# Autodesk Inventor assembly: Koło_przednie
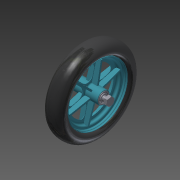
[picture p0: Inventor's stored thumbnail of the model, 180x180]
Saved by Autodesk Inventor 2015 (Build 190159000, 159)
## iProperties
Created: 2015-12-01
Part Number: Koło_przednie
Document SubType Name: Assembly
Designer: graaapsik
Author: graaapsik
## Documents named in this file (7)
- C:\Users\EriveltonDell\Documents\Centro Universitário da FEI\Wheelchair\CADEIRA DE RODAS - DESENHO\lasteverision\Power-Assisted-Wheelchair-master\Koło_przednie.iam
- C:\Users\EriveltonDell\Documents\Centro Universitário da FEI\Wheelchair\CADEIRA DE RODAS - DESENHO\lasteverision\Power-Assisted-Wheelchair-master\Obręcz_koła_przedniego.ipt
- C:\Users\EriveltonDell\Documents\Centro Universitário da FEI\Wheelchair\CADEIRA DE RODAS - DESENHO\lasteverision\Power-Assisted-Wheelchair-master\ISO 4016 - M8 x 65.ipt
- C:\Users\EriveltonDell\Documents\Centro Universitário da FEI\Wheelchair\CADEIRA DE RODAS - DESENHO\lasteverision\Power-Assisted-Wheelchair-master\ISO 4032 - M8ISO.ipt
- C:\Users\EriveltonDell\Documents\Centro Universitário da FEI\Wheelchair\CADEIRA DE RODAS - DESENHO\lasteverision\Power-Assisted-Wheelchair-master\Rolling bearing 70000B S719_8 GB_T 292-94.ipt
- C:\Users\EriveltonDell\Documents\Centro Universitário da FEI\Wheelchair\CADEIRA DE RODAS - DESENHO\lasteverision\Power-Assisted-Wheelchair-master\Separator.ipt
- C:\Users\EriveltonDell\Documents\Centro Universitário da FEI\Wheelchair\CADEIRA DE RODAS - DESENHO\lasteverision\Power-Assisted-Wheelchair-master\Opona_koła_przedniego.ipt
## Components (11 placed, 6 different names)
1. Separator:1 — Zestawiający:6, Zestawiający:7, Zestawiający:8, Walcowe:2, Wstaw:1, Wstaw:3
2. Obręcz_koła_przedniego:1 — Walcowe:1, Walcowe:2, Równoległy:3
3. Opona_koła_przedniego:1 — Równoległy:3
4. ISO 4016 M8 x 65:1 — Walcowe:1, Zestawiający:1, Zestawiający:2, Zestawiający:3, Zestawiający:4, Zestawiający:6
5. Rolling bearing GB/T 292-2007 Type 70000B S719/8:1 — Zestawiający:1, Zestawiający:4, Zestawiający:7, Symetria:1
6. Rolling bearing GB/T 292-2007 Type 70000B S719/8:2 — Zestawiający:2, Zestawiający:5, Zestawiający:8, Symetria:1
7. ISO 4032 M8:1 — Zestawiający:3, Zestawiający:5
8. ISO 4016 M8 x 65:2 — Zestawiający:9, Zestawiający:10, Zestawiający:11
9. ISO 4032 M8:2 — Zestawiający:11, Zestawiający:12
10. Rolling bearing GB/T 292-2007 Type 70000B S719/8:3 — Wstaw:3, Zestawiający:12
11. Rolling bearing GB/T 292-2007 Type 70000B S719/8:4 — Wstaw:1, Zestawiający:9, Zestawiający:10
## Relationships (18: Mate 12, CylindricalJoint 2, Insert 2, Symmetry 1, Flush 1)
- Walcowe:1 [CylindricalJoint]: Obręcz_koła_przedniego:1 ↔ ISO 4016 M8 x 65:1
- Zestawiający:1 [Mate]: ISO 4016 M8 x 65:1 ↔ Rolling bearing GB/T 292-2007 Type 70000B S719/8:1
- Zestawiający:2 [Mate]: ISO 4016 M8 x 65:1 ↔ Rolling bearing GB/T 292-2007 Type 70000B S719/8:2
- Zestawiający:3 [Mate]: ISO 4016 M8 x 65:1 ↔ ISO 4032 M8:1
- Zestawiający:4 [Mate] (6 mm): ISO 4016 M8 x 65:1 ↔ Rolling bearing GB/T 292-2007 Type 70000B S719/8:1
- Zestawiający:5 [Mate] (6 mm): Rolling bearing GB/T 292-2007 Type 70000B S719/8:2 ↔ ISO 4032 M8:1
- Zestawiający:6 [Mate]: Separator:1 ↔ ISO 4016 M8 x 65:1
- Zestawiający:7 [Mate]: Separator:1 ↔ Rolling bearing GB/T 292-2007 Type 70000B S719/8:1
- Zestawiający:8 [Mate]: Separator:1 ↔ Rolling bearing GB/T 292-2007 Type 70000B S719/8:2
- Walcowe:2 [CylindricalJoint]: Separator:1 ↔ Obręcz_koła_przedniego:1
- Symetria:1 [Symmetry]: Rolling bearing GB/T 292-2007 Type 70000B S719/8:1 ↔ Rolling bearing GB/T 292-2007 Type 70000B S719/8:2
- Równoległy:3 [Flush]: Obręcz_koła_przedniego:1 ↔ Opona_koła_przedniego:1
- Wstaw:1 [Insert]: Separator:1 ↔ Rolling bearing GB/T 292-2007 Type 70000B S719/8:4
- Wstaw:3 [Insert]: Separator:1 ↔ Rolling bearing GB/T 292-2007 Type 70000B S719/8:3
- Zestawiający:9 [Mate]: ISO 4016 M8 x 65:2 ↔ Rolling bearing GB/T 292-2007 Type 70000B S719/8:4
- Zestawiający:10 [Mate] (6 mm): ISO 4016 M8 x 65:2 ↔ Rolling bearing GB/T 292-2007 Type 70000B S719/8:4
- Zestawiający:11 [Mate]: ISO 4016 M8 x 65:2 ↔ ISO 4032 M8:2
- Zestawiający:12 [Mate] (6 mm): ISO 4032 M8:2 ↔ Rolling bearing GB/T 292-2007 Type 70000B S719/8:3
